# Autodesk Inventor assembly: Roda
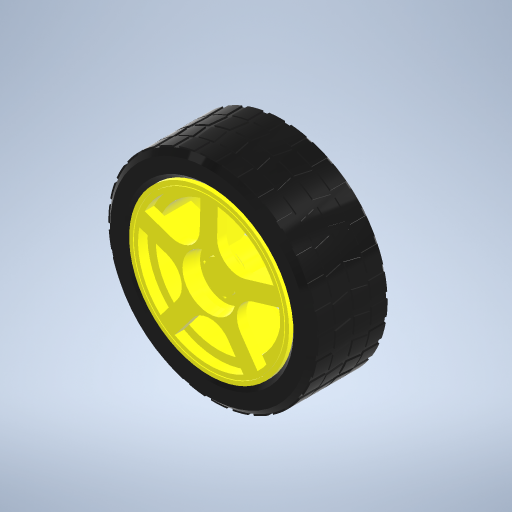
[picture p0: Inventor's stored thumbnail of the model, 512x512]
Saved by Autodesk Inventor 2023 (Build 270158000, 158)
## iProperties
Created: 2023-08-31
Part Number: Roda
Document SubType Name: Assembly
Designer: LENOVO IP320-14IKB
Author: LENOVO IP320-14IKB
## Documents named in this file (3)
- D:\Backup C\Documents\Inventor\PMLDCAPSTONE\RODA\Roda.iam
- D:\Backup C\Documents\Inventor\PMLDCAPSTONE\RODA\Karet Roda Mainan.ipt
- D:\Backup C\Documents\Inventor\PMLDCAPSTONE\RODA\Velg Roda Mainan.ipt
## Components (2 placed, 2 different names)
1. Karet Roda Mainan:1 — Rotational:3
2. Velg Roda Mainan:1 — Mate:1, Mate:2, Rotational:3
## Relationships (3: Mate 2, RevoluteJoint 1)
- Mate:1: Velg Roda Mainan:1
- Mate:2: Velg Roda Mainan:1
- Rotational:3 [RevoluteJoint]: Karet Roda Mainan:1 ↔ Velg Roda Mainan:1
